# Autodesk Inventor assembly: _pumpswitch_top
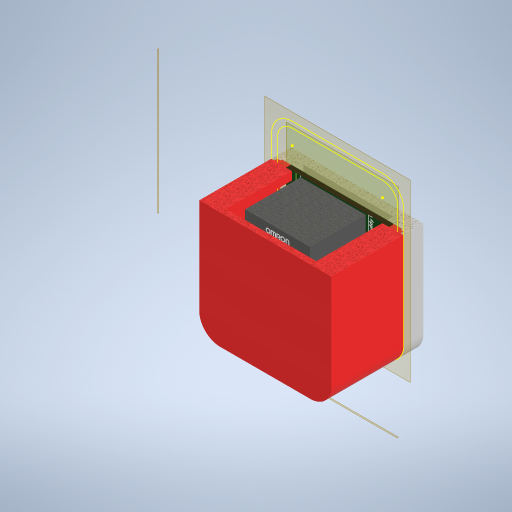
[picture p0: Inventor's stored thumbnail of the model, 512x512]
Saved by Autodesk Inventor 2024.3 (Build 283343000, 343)
## iProperties
Created: 2024-10-21
Part Number: _pumpswitch_top
Document SubType Name: Assembly
Designer: atrus
Author: atrus
## Documents named in this file (4)
- C:\Users\atrus\Dropbox\elec\Mechanical\osmoBuddy\_pumpswitch_top.iam
- C:\Users\atrus\Dropbox\elec\Mechanical\osmoBuddy\PCB_PumpSwitch\osmobuddy_pumpswitch_v1.iam
- C:\Users\atrus\Dropbox\elec\Mechanical\osmoBuddy\pumpswitch_bottom.ipt
- C:\Users\atrus\Dropbox\elec\Mechanical\osmoBuddy\pumpswitch_top.ipt
## Components (3 placed, 3 different names)
1. osmobuddy_pumpswitch_v1:1 [sub-assembly] — Flush:1, Flush:2
2. pumpswitch_bottom:1 — Flush:1, Flush:2, Flush:3, Flush:4
3. pumpswitch_top:1 — Flush:3, Flush:4
## Relationships (4: Flush 4)
- Flush:1: osmobuddy_pumpswitch_v1:1 ↔ pumpswitch_bottom:1
- Flush:2: osmobuddy_pumpswitch_v1:1 ↔ pumpswitch_bottom:1
- Flush:3: pumpswitch_bottom:1 ↔ pumpswitch_top:1
- Flush:4: pumpswitch_bottom:1 ↔ pumpswitch_top:1
